# Autodesk Inventor assembly: FINAL-ASM
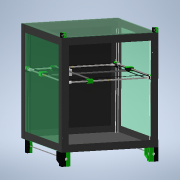
[picture p0: Inventor's stored thumbnail of the model, 180x180]
Saved by Autodesk Inventor 2020.4 (Build 244396000, 396)
## iProperties
Created: 2021-03-10
Part Number: FINAL-ASM
Document SubType Name: Assembly
Designer: AOB
Mass: 12460.3 g
Surface Area: 42719.4 cm^2
Volume: 5012.57 cm^3
Density: 2.48581 g/cm^3
Author: AOB
## Documents named in this file (10)
- C:\Users\marti\Documents\Inventor\ProjectBoron\Boron Ultima\Boron Ultima.iam
- C:\Users\marti\Documents\Inventor\ProjectBoron\Boron Ultima\frame.iam
- C:\Users\marti\Documents\Inventor\ProjectBoron\Boron Ultima\Zmotionassembly.iam
- C:\Users\marti\Documents\Inventor\ProjectBoron\Boron Ultima\Zmotionassembly(right)1.iam
- C:\Users\marti\Documents\Inventor\ProjectBoron\Boron Ultima\xy-motion-assembly.iam
- C:\Users\marti\Documents\Inventor\ProjectBoron\Boron Ultima\side panel.ipt
- C:\Users\marti\Documents\Inventor\ProjectBoron\Boron Ultima\top-idler.iam
- C:\Users\marti\Documents\Inventor\ProjectBoron\Boron Ultima\back cover.ipt
- C:\Users\marti\Documents\Inventor\ProjectBoron\Boron Ultima\toppanel.ipt
- C:\Users\marti\Documents\Inventor\ProjectBoron\Boron Ultima\bottom panel.ipt
## Components (11 placed, 9 different names)
1. frame:1 [sub-assembly] — Mate:1, Flush:1, Flush:2, Symmetry:1, Mate:2, Flush:4, Flush:5, Mate:8, Mate:9, Mate:11, Rigid:1, Rigid:2, Mate:10, Mate:13, Flush:13, Flush:16, Flush:15, Mate:14, Mate:18, Mate:19
2. Zmotionassembly:2 [sub-assembly] — Mate:1, Flush:1, Flush:2, Symmetry:1
3. Zmotionassembly(right)1:1 [sub-assembly] — Mate:2, Flush:4, Flush:5, Mate:7
4. xy-motion-assembly:1 [sub-assembly] — Mate:7, Flush:7
5. side panel:1 — Mate:8, Mate:9, Mate:17
6. side panel:2 — Mate:10, Mate:11
7. top-idler:1 [sub-assembly] — Rigid:2
8. top-idler:2 [sub-assembly] — Rigid:1
9. back cover:1 — Mate:13, Flush:13
10. toppanel:1 — Flush:16, Flush:15, Mate:14
11. bottom panel:1 — Mate:17, Mate:18, Mate:19
## Relationships (23: Mate 12, Flush 8, WeldJoint 2, Symmetry 1)
- Mate:1: frame:1 ↔ Zmotionassembly:2
- Flush:1: frame:1 ↔ Zmotionassembly:2
- Flush:2: frame:1 ↔ Zmotionassembly:2
- Symmetry:1: frame:1 ↔ Zmotionassembly:2
- Mate:2: frame:1 ↔ Zmotionassembly(right)1:1
- Flush:4: frame:1 ↔ Zmotionassembly(right)1:1
- Flush:5: frame:1 ↔ Zmotionassembly(right)1:1
- Mate:7 (1 mm): Zmotionassembly(right)1:1 ↔ xy-motion-assembly:1
- Flush:7: xy-motion-assembly:1
- Mate:8: frame:1 ↔ side panel:1
- Mate:9 (5 mm): frame:1 ↔ side panel:1
- Mate:10 (5 mm): frame:1 ↔ side panel:2
- Mate:11 (5 mm): frame:1 ↔ side panel:2
- Rigid:1 [WeldJoint]: frame:1 ↔ top-idler:2
- Rigid:2 [WeldJoint]: frame:1 ↔ top-idler:1
- Flush:13: frame:1 ↔ back cover:1
- Mate:13: frame:1 ↔ back cover:1
- Flush:16: frame:1 ↔ toppanel:1
- Flush:15: frame:1 ↔ toppanel:1
- Mate:14: frame:1 ↔ toppanel:1
- Mate:17: side panel:1 ↔ bottom panel:1
- Mate:18: frame:1 ↔ bottom panel:1
- Mate:19: frame:1 ↔ bottom panel:1
